# Autodesk Inventor assembly: CNC Layout
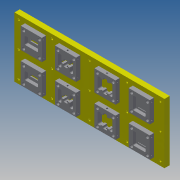
[picture p0: Inventor's stored thumbnail of the model, 180x180]
Saved by Autodesk Inventor 2015 (Build 190159000, 159)
## iProperties
Created: 2014-10-08
Part Number: CNC Layout
Document SubType Name: Assembly
Designer: jdyne
Author: jdyne
## Documents named in this file (6)
- D:\Documents\Inventor\Microwave Transmission line\CNC Layout.iam
- D:\Documents\Inventor\Microwave Transmission line\CNC Assembly.ipt
- D:\Documents\Inventor\Microwave Transmission line\Holder.ipt
- D:\Documents\Inventor\Microwave Transmission line\HolderEnd.ipt
- D:\Documents\Inventor\Microwave Transmission line\HolderStart.ipt
- D:\Documents\Inventor\Microwave Transmission line\HolderThin2.ipt
## Components (9 placed, 5 different names)
1. CNC Assembly:1 — Mate:1, Mate:2, Mate:3, Mate:4, Mate:5, Mate:6, Mate:7, Mate:8, Flush:2, Flush:3, Flush:4, Flush:6, Flush:7, Flush:8, Flush:9, Flush:13, Flush:14, Flush:15, Flush:16, Flush:17, Flush:18, Flush:19, Flush:20, Flush:21
2. Holder:1 — Mate:5, Flush:2, Flush:14
3. Holder:2 — Mate:6, Flush:7, Flush:13
4. HolderEnd:1 — Mate:7, Flush:18, Flush:21
5. HolderEnd:2 — Mate:8, Flush:8, Flush:19
6. HolderStart:1 — Mate:1, Flush:17, Flush:20
7. HolderStart:2 — Mate:2, Flush:4, Flush:9
8. HolderThin2:1 — Mate:3, Flush:3, Flush:15
9. HolderThin2:2 — Mate:4, Flush:6, Flush:16
## Relationships (24: Flush 16, Mate 8)
- Mate:1: CNC Assembly:1 ↔ HolderStart:1
- Mate:2: CNC Assembly:1 ↔ HolderStart:2
- Mate:3: CNC Assembly:1 ↔ HolderThin2:1
- Mate:4: CNC Assembly:1 ↔ HolderThin2:2
- Mate:5: CNC Assembly:1 ↔ Holder:1
- Mate:6: CNC Assembly:1 ↔ Holder:2
- Mate:7: CNC Assembly:1 ↔ HolderEnd:1
- Mate:8: CNC Assembly:1 ↔ HolderEnd:2
- Flush:2 (-8 mm): CNC Assembly:1 ↔ Holder:1
- Flush:3 (-8 mm): CNC Assembly:1 ↔ HolderThin2:1
- Flush:4 (8 mm): CNC Assembly:1 ↔ HolderStart:2
- Flush:6 (-8 mm): CNC Assembly:1 ↔ HolderThin2:2
- Flush:7 (-8 mm): CNC Assembly:1 ↔ Holder:2
- Flush:8 (-8 mm): CNC Assembly:1 ↔ HolderEnd:2
- Flush:9 (20 mm): CNC Assembly:1 ↔ HolderStart:2
- Flush:13 (85 mm): CNC Assembly:1 ↔ Holder:2
- Flush:14 (85 mm): CNC Assembly:1 ↔ Holder:1
- Flush:15 (-85 mm): CNC Assembly:1 ↔ HolderThin2:1
- Flush:16 (85 mm): CNC Assembly:1 ↔ HolderThin2:2
- Flush:17 (-8 mm): CNC Assembly:1 ↔ HolderStart:1
- Flush:18 (-8 mm): CNC Assembly:1 ↔ HolderEnd:1
- Flush:19 (-20 mm): CNC Assembly:1 ↔ HolderEnd:2
- Flush:20 (-20 mm): CNC Assembly:1 ↔ HolderStart:1
- Flush:21 (20 mm): CNC Assembly:1 ↔ HolderEnd:1
